# Autodesk Inventor assembly: Primary_cover_presentation
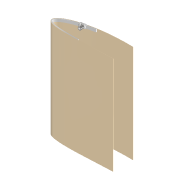
[picture p0: Inventor's stored thumbnail of the model, 180x180]
Saved by Autodesk Inventor 2022 (Build 260153000, 153)
## iProperties
Created: 2022-10-12
Part Number: Primary_cover_presentation
Document SubType Name: Assembly
Designer: dell
Author: dell
## Documents named in this file (4)
- D:\xxxx\Uni\Part IV\MECHENG_700\Part_IV_project_CAD\Bird_skeleton_prototypes\Wing_drone_V1\Bird_wing_V2\Wing_cover\Primary_cover_presentation.iam
- D:\xxxx\Uni\Part IV\MECHENG_700\Part_IV_project_CAD\Bird_skeleton_prototypes\Wing_drone_V1\Bird_wing_V2\Wing_cover\Radius_joint_cover_film_V2.ipt
- D:\xxxx\Uni\Part IV\MECHENG_700\Part_IV_project_CAD\Bird_skeleton_prototypes\Wing_drone_V1\Bird_wing_V2\Wing_cover\Radius_joint_cover_V2.ipt
- D:\xxxx\Uni\Part IV\MECHENG_700\Part_IV_project_CAD\Bird_skeleton_prototypes\Wing_drone_V1\Bird_wing_V2\Wing_cover\Torsion_spring.ipt
## Components (3 placed, 3 different names)
1. Radius_joint_cover_film_V2:1 — Flush:1
2. Radius_joint_cover_V2:1 — Flush:1, Mate:1, Mate:2
3. Torsion_spring:1 — Mate:1, Mate:2
## Relationships (3: Mate 2, Flush 1)
- Flush:1: Radius_joint_cover_film_V2:1 ↔ Radius_joint_cover_V2:1
- Mate:1: Radius_joint_cover_V2:1 ↔ Torsion_spring:1
- Mate:2: Radius_joint_cover_V2:1 ↔ Torsion_spring:1
